# Autodesk Inventor assembly: Assembly
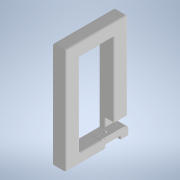
[picture p0: Inventor's stored thumbnail of the model, 180x180]
Saved by Autodesk Inventor 2020.1 (Build 241239000, 239)
## iProperties
Created: 2022-04-03
Part Number: Assembly
Document SubType Name: Assembly
Designer: OEM
Author: OEM
## Documents named in this file (3)
- C:\Users\OEM\Desktop\HandSomething\Drzwi_CAD\Assembly.iam
- C:\Users\OEM\Desktop\HandSomething\Drzwi_CAD\Framuga.ipt
- C:\Users\OEM\Desktop\HandSomething\Drzwi_CAD\servo_sub.ipt
## Components (2 placed, 2 different names)
1. Framuga:2 — Mate:1, Mate:2, Mate:3
2. servo_sub:2 — Mate:1, Mate:2, Mate:3
## Relationships (3: Mate 3)
- Mate:1: Framuga:2 ↔ servo_sub:2
- Mate:2: Framuga:2 ↔ servo_sub:2
- Mate:3: Framuga:2 ↔ servo_sub:2
